# Autodesk Inventor assembly: Motor
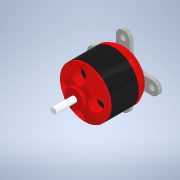
[picture p0: Inventor's stored thumbnail of the model, 180x180]
Saved by Autodesk Inventor 2020 (Build 240168000, 168)
## iProperties
Created: 2019-06-13
Part Number: Motor
Document SubType Name: Assembly
Designer: amirt
Author: amirt
## Documents named in this file (3)
- C:\Users\amirt\Documents\Inventor\Drone\Motor.iam
- C:\Users\amirt\Documents\Inventor\Drone\Motor\BR2212 Mount v1.ipt
- C:\Users\amirt\Documents\Inventor\Drone\Motor\BR2212 Body v1.ipt
## Components (2 placed, 2 different names)
1. BR2212 Mount v1:1 — Insert:1, Insert:2, Mate:1
2. BR2212 Body v1:1 — Insert:1, Insert:2, Mate:1
## Relationships (3: Insert 2, Mate 1)
- Insert:1: BR2212 Mount v1:1 ↔ BR2212 Body v1:1
- Insert:2: BR2212 Mount v1:1 ↔ BR2212 Body v1:1
- Mate:1: BR2212 Mount v1:1 ↔ BR2212 Body v1:1
